# Autodesk Inventor assembly: ASY 000 ДМФ Disk Micro filter v3.0
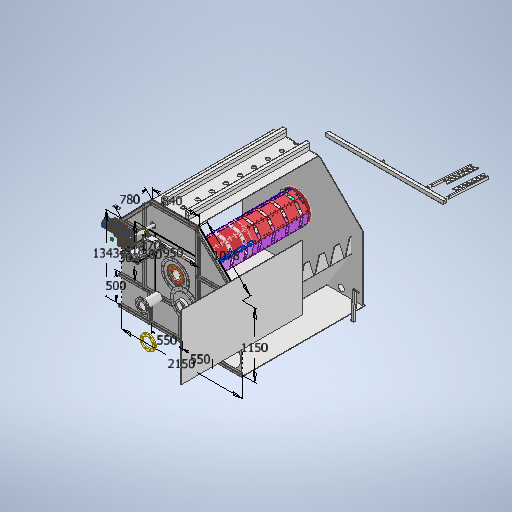
[picture p0: Inventor's stored thumbnail of the model, 512x512]
Saved by Autodesk Inventor 2026.2 (Build 302298000, 298)
## iProperties
Part Number: ASY 000 ДМФ Disk Micro filter v3.0
Document SubType Name: Assembly
Designer: admin
Author: admin
## Documents named in this file (35)
- C:\Users\admin\Documents\Inventor\DMF-Disk-Micro-Filter\ASY 000 ДМФ Disk Micro filter v3.0.iam
- C:\Users\admin\Documents\Inventor\DMF-Disk-Micro-Filter\Wall right v2.0.ipt
- C:\Users\admin\Documents\Inventor\DMF-Disk-Micro-Filter\DF1.03 Wall bottom v2.0.ipt
- C:\Users\admin\Documents\Inventor\DMF-Disk-Micro-Filter\DF1.04 Wall face v2.0.ipt
- C:\Users\admin\Documents\Inventor\DMF-Disk-Micro-Filter\ДМФ 093 Постель КОРМА v2.0.ipt
- C:\Users\admin\Documents\Inventor\DMF-Disk-Micro-Filter\ДМФ 055 труба илоотвода v2.0.ipt
- C:\Users\admin\Documents\Inventor\DMF-Disk-Micro-Filter\ДМФ 033 держатель лотка v2.0.ipt
- C:\Users\admin\Documents\Inventor\DMF-Disk-Micro-Filter\ASY ДМФ лоток 050 илоотвод v2.0.iam
- C:\Users\admin\Documents\Inventor\DMF-Disk-Micro-Filter\ДМФ 066 Гребенка v2.0.ipt
- C:\Users\admin\Documents\Inventor\DMF-Disk-Micro-Filter\ДМФ 067 крышка v2.0.ipt
- C:\Users\admin\Documents\Inventor\DMF-Disk-Micro-Filter\ДМФ 081 труба форсунки v2.0.ipt
- C:\Users\admin\Documents\Inventor\DMF-Disk-Micro-Filter\ASY Обрешетка лицевая стенка.iam
- C:\Users\admin\Documents\Inventor\DMF-Disk-Micro-Filter\Вал ведущей шестерни.ipt
- C:\Users\admin\Documents\Inventor\DMF-Disk-Micro-Filter\Корпусный подшипник D35.ipt
- C:\Users\admin\Documents\Inventor\DMF-Disk-Micro-Filter\Мотор-редуктор NMRV 090(80B5).ipt
- C:\Users\admin\Documents\Inventor\DMF-Disk-Micro-Filter\DMF pancake.ipt
- C:\Users\admin\Documents\Inventor\DMF-Disk-Micro-Filter\Нога для постели №2.ipt
- C:\Users\admin\Documents\Inventor\DMF-Disk-Micro-Filter\ДМФ 094 Постель НОС крепление v2.0.ipt
- C:\Users\admin\Documents\Inventor\DMF-Disk-Micro-Filter\DMF Hat 2.0.ipt
- C:\Users\admin\Documents\Inventor\DMF-Disk-Micro-Filter\DMF Flange exit 2.0.ipt
- C:\Users\admin\Documents\Inventor\DMF-Disk-Micro-Filter\Барабан v2.1\ASY ДМФ 0100 Барабан v2.1.iam
- C:\Users\admin\Documents\Inventor\DMF-Disk-Micro-Filter\Барабан v2.1\DMF flange small gear.ipt
- C:\Users\admin\Documents\Inventor\DMF-Disk-Micro-Filter\Барабан v2.1\DMF small gear.ipt
- C:\Users\admin\Documents\Inventor\DMF-Disk-Micro-Filter\DMF Support ring tail.ipt
- C:\Users\admin\Documents\Inventor\DMF-Disk-Micro-Filter\DMF 082 коллектор болванка.ipt
- C:\Users\admin\Documents\Inventor\DMF-Disk-Micro-Filter\Барабан v2.1\DMF 2.1 Пластина паза маленькая.ipt
- C:\Users\admin\Documents\Inventor\DMF-Disk-Micro-Filter\Барабан v2.1\DMF 2.1 01 45 Gear ring 5.ipt
- C:\Users\admin\Documents\Inventor\DMF-Disk-Micro-Filter\ДМФ 01 15 Барабан усилитель борта.ipt
- C:\Users\admin\Documents\Inventor\DMF-Disk-Micro-Filter\ДМФ 01 15 Барабан усилитель борта_CPY.ipt
- C:\Users\admin\Documents\Inventor\DMF-Disk-Micro-Filter\Барабан v2.1\DMF flange small gear 2.ipt
- C:\Users\admin\Documents\Inventor\DMF-Disk-Micro-Filter\Left wall v2.0.ipt
- C:\Users\admin\Documents\Inventor\DMF-Disk-Micro-Filter\Барабан v2.1\DMF 01 31 Барабан Опорное кольцо НОС v2.1.ipt
- C:\Users\admin\Documents\Inventor\DMF-Disk-Micro-Filter\Подставка под мотор.iam
- C:\Users\admin\Documents\Inventor\DMF-Disk-Micro-Filter\Барабан v2.1\DMF 2.1 01 45 Gear ring 5_CPY.ipt
- C:\Users\admin\Documents\Inventor\DMF-Disk-Micro-Filter\ДМФ 093 Постель КОРМА v2.0_CPY.ipt
## Components (36 placed, 34 different names)
1. ASY ДМФ 0100 Барабан v2.1:1 [sub-assembly]
2. ASY ДМФ лоток 050 илоотвод v2.0:1 [sub-assembly] — Rigid:14
3. ASY Обрешетка лицевая стенка:1 [sub-assembly] — Mate:13, Flush:5, Flush:6
4. Wall right v2.0:1 — Rigid:8, Mate:14, Rigid:12
5. DMF Support ring tail:1
6. Left wall v2.0:1 — Rigid:9, Mate:13, Flush:5, Flush:6, Flush:7, Mate:15, Flush:8, Rotational:4, Rigid:10
7. DF1.03 Wall bottom v2.0:1 — Mate:10, Mate:11, Rigid:8, Mate:12, Rigid:9, Mate:16
8. DF1.04 Wall face v2.0:1
9. DMF 2.1 01 45 Gear ring 5:1 — Rigid:10, Rigid:11, Rigid:14
10. ДМФ 093 Постель КОРМА v2.0:1 — Rigid:11
11. ДМФ 055 труба илоотвода v2.0:1
12. ДМФ 033 держатель лотка v2.0:1
13. ДМФ 066 Гребенка v2.0:1 — Mate:15, Flush:8, Mate:16
14. ДМФ 067 крышка v2.0:1 — Mate:14, Flush:7
15. ДМФ 081 труба форсунки v2.0:1
16. Вал ведущей шестерни:1 — Rotational:5
17. Корпусный подшипник D35:1 — Angle:1, Mate:19
18. Мотор-редуктор NMRV 090(80B5):1 — Rotational:5, Angle:1
19. DMF pancake:1
20. Нога для постели №2:1 — Mate:18, Flush:9
21. ДМФ 094 Постель НОС крепление v2.0:1
22. DMF Hat 2.0:1
23. DMF Flange exit 2.0:1
24. flange small gear:1
25. DMF small gear:1 — Rotational:4
26. DMF 082 коллектор болванка:1
27. ДМФ 081 труба форсунки v2.0:2
28. DMF 2.1 Пластина паза маленькая:1
29. ДМФ 01 15 Барабан усилитель борта:1
30. ДМФ 01 15 Барабан усилитель борта_CPY:1
31. DMF flange small gear 2:1
32. DMF 01 31 Барабан Опорное кольцо НОС v2.1:1
33. ДМФ 094 Постель НОС крепление v2.0:2
34. Подставка под мотор:1 [sub-assembly] — Mate:18, Mate:19, Flush:9
35. DMF 2.1 01 45 Gear ring 5_CPY:1 — Rigid:12, Rigid:13
36. ДМФ 093 Постель КОРМА v2.0_CPY:1 — Rigid:13
## Relationships (39: WeldJoint 14, Mate 12, Flush 7, RevoluteJoint 5, Angle 1)
- [WeldJoint]: ДМФ 055 труба илоотвода v2.0:1 ↔ DMF Flange exit 2.0:1
- [WeldJoint]: DMF pancake:1 ↔ DMF Hat 2.0:1
- [WeldJoint]: Wall right v2.0:1 ↔ DMF Support ring tail:1
- [RevoluteJoint]: ASY ДМФ 0100 Барабан v2.1:1 ↔ DMF Support ring tail:1
- [RevoluteJoint]: ASY ДМФ 0100 Барабан v2.1:1 ↔ DMF Support ring tail:1
- [WeldJoint]: ДМФ 081 труба форсунки v2.0:1 ↔ DMF 082 коллектор болванка:1
- [WeldJoint]: DMF 082 коллектор болванка:1 ↔ ДМФ 081 труба форсунки v2.0:2
- [Mate]: DMF 082 коллектор болванка:1 ↔ ДМФ 01 15 Барабан усилитель борта:1
- [Mate]: DMF 082 коллектор болванка:1 ↔ ДМФ 01 15 Барабан усилитель борта:1
- [Flush]: ДМФ 033 держатель лотка v2.0:1 ↔ ДМФ 01 15 Барабан усилитель борта_CPY:1
- [RevoluteJoint]: Вал ведущей шестерни:1 ↔ DMF small gear:1
- [WeldJoint]: flange small gear:1 ↔ DMF flange small gear 2:1
- [WeldJoint] (-25 mm): Вал ведущей шестерни:1 ↔ flange small gear:1
- [Flush]: ASY Обрешетка лицевая стенка:1 ↔ Нога для постели №2:1
- [Mate]: ASY Обрешетка лицевая стенка:1 ↔ Нога для постели №2:1
- Mate:10: DF1.03 Wall bottom v2.0:1
- Mate:11: DF1.03 Wall bottom v2.0:1
- Rigid:8 [WeldJoint] (-25 mm): Wall right v2.0:1 ↔ DF1.03 Wall bottom v2.0:1
- Mate:12: DF1.03 Wall bottom v2.0:1
- Rigid:9 [WeldJoint] (-25 mm): Left wall v2.0:1 ↔ DF1.03 Wall bottom v2.0:1
- Mate:13: ASY Обрешетка лицевая стенка:1 ↔ Left wall v2.0:1
- Flush:5: ASY Обрешетка лицевая стенка:1 ↔ Left wall v2.0:1
- Flush:6: ASY Обрешетка лицевая стенка:1 ↔ Left wall v2.0:1
- Mate:14: Wall right v2.0:1 ↔ ДМФ 067 крышка v2.0:1
- Flush:7: Left wall v2.0:1 ↔ ДМФ 067 крышка v2.0:1
- Mate:15: Left wall v2.0:1 ↔ ДМФ 066 Гребенка v2.0:1
- Flush:8 (200 mm): Left wall v2.0:1 ↔ ДМФ 066 Гребенка v2.0:1
- Mate:16: DF1.03 Wall bottom v2.0:1 ↔ ДМФ 066 Гребенка v2.0:1
- Rotational:4 [RevoluteJoint] (-33 mm): Left wall v2.0:1 ↔ DMF small gear:1
- Rotational:5 [RevoluteJoint] (3 mm): Вал ведущей шестерни:1 ↔ Мотор-редуктор NMRV 090(80B5):1
- Rigid:10 [WeldJoint]: Left wall v2.0:1 ↔ DMF 2.1 01 45 Gear ring 5:1
- Rigid:11 [WeldJoint]: DMF 2.1 01 45 Gear ring 5:1 ↔ ДМФ 093 Постель КОРМА v2.0:1
- Angle:1 (0 deg): Корпусный подшипник D35:1 ↔ Мотор-редуктор NMRV 090(80B5):1
- Mate:18: Нога для постели №2:1 ↔ Подставка под мотор:1
- Mate:19: Корпусный подшипник D35:1 ↔ Подставка под мотор:1
- Flush:9: Нога для постели №2:1 ↔ Подставка под мотор:1
- Rigid:12 [WeldJoint]: Wall right v2.0:1 ↔ DMF 2.1 01 45 Gear ring 5_CPY:1
- Rigid:13 [WeldJoint]: DMF 2.1 01 45 Gear ring 5_CPY:1 ↔ ДМФ 093 Постель КОРМА v2.0_CPY:1
- Rigid:14 [WeldJoint]: ASY ДМФ лоток 050 илоотвод v2.0:1 ↔ DMF 2.1 01 45 Gear ring 5:1
